# Autodesk Inventor assembly: Camera
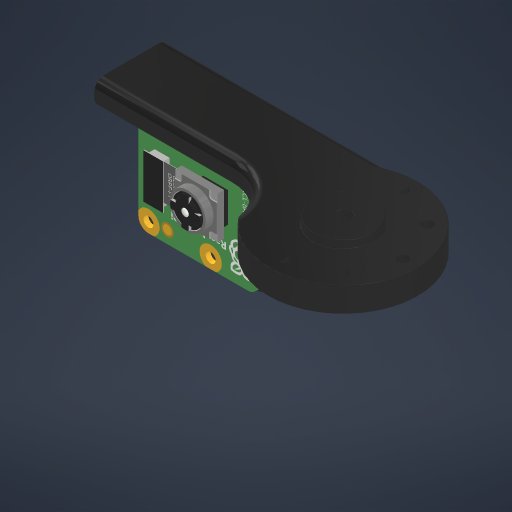
[picture p0: Inventor's stored thumbnail of the model, 512x512]
Saved by Autodesk Inventor 2023 (Build 270158000, 158)
## iProperties
Created: 2023-04-13
Part Number: Camera
Document SubType Name: Assembly
Designer: vatdu
Author: vatdu
## Documents named in this file (3)
- C:\Users\vatdu\Desktop\CRYSTAL MARK II\Components\Camera.iam
- C:\Users\vatdu\Desktop\CRYSTAL MARK II\Components\Camera Mount.ipt
- C:\Users\vatdu\Desktop\CRYSTAL MARK II\Components\Raspberry Pi Camera.ipt
## Components (2 placed, 2 different names)
1. Camera Mount:1 — Rotational:1
2. Raspberry Pi Camera:1 — Rotational:1
## Relationships (1: RevoluteJoint 1)
- Rotational:1 [RevoluteJoint]: Camera Mount:1 ↔ Raspberry Pi Camera:1
